# Autodesk Inventor assembly: DoubleCross_Rturn
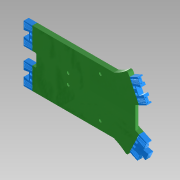
[picture p0: Inventor's stored thumbnail of the model, 180x180]
Saved by Autodesk Inventor 2021 (Build 250183000, 183)
## iProperties
Created: 2021-03-02
Part Number: DoubleCross_Rturn
Document SubType Name: Assembly
Designer: kumagai
Author: kumagai
## Documents named in this file (9)
- X:\Develop\CAD\PlaRails\DoubleCross\DoubleCross_SymWiden.iam
- X:\Develop\CAD\PlaRails\DoubleCross\DoubleCross\DoubleCross-ST_R.ipt
- Z:\Develop\CAD\PlaRails\DoubleCross.ipt
- X:\Develop\CAD\PlaRails\DoubleCross\DoubleCross\DoubleCross-ST_M.ipt
- X:\Develop\CAD\PlaRails\RailJointFemale.ipt
- X:\Develop\CAD\PlaRails\DoubleCross\DoubleCross\DoubleCross-SL_M.ipt
- X:\Develop\CAD\PlaRails\DoubleCross\DoubleCross.ipt
- X:\Develop\CAD\PlaRails\DoubleCross\DoubleCross\DoubleCross-SL_R.ipt
- X:\Develop\CAD\PlaRails\RailJointMale.ipt
## Components (8 placed, 6 different names)
1. Rail_LF — メイト:6, フラッシュ:12, フラッシュ:18
2. Rail_RF — メイト:5, フラッシュ:26, フラッシュ:15, フラッシュ:22, フラッシュ:23, フラッシュ:19
3. Rail_LB — フラッシュ:9, メイト:7, フラッシュ:11, フラッシュ:16, フラッシュ:20, フラッシュ:21
4. Rail_RB — フラッシュ:7, メイト:4, フラッシュ:14, フラッシュ:17, フラッシュ:24, フラッシュ:25
5. RailJointFemale:4 — メイト:5, フラッシュ:26, フラッシュ:19
6. RailJointMale:1 — フラッシュ:7, メイト:4, フラッシュ:14
7. RailJointFemale:1 — メイト:6, フラッシュ:12, フラッシュ:18
8. RailJointFemale:2 — フラッシュ:9, メイト:7, フラッシュ:11
## Relationships (21: Flush 17, Mate 4)
- フラッシュ:7 [Flush]: Rail_RB ↔ RailJointMale:1
- フラッシュ:9 [Flush]: Rail_LB ↔ RailJointFemale:2
- メイト:4 [Mate]: Rail_RB ↔ RailJointMale:1
- メイト:5 [Mate]: Rail_RF ↔ RailJointFemale:4
- メイト:6 [Mate]: Rail_LF ↔ RailJointFemale:1
- メイト:7 [Mate]: Rail_LB ↔ RailJointFemale:2
- フラッシュ:11 [Flush]: Rail_LB ↔ RailJointFemale:2
- フラッシュ:12 [Flush]: Rail_LF ↔ RailJointFemale:1
- フラッシュ:26 [Flush]: Rail_RF ↔ RailJointFemale:4
- フラッシュ:14 [Flush]: Rail_RB ↔ RailJointMale:1
- フラッシュ:15 [Flush]: Rail_RF
- フラッシュ:22 [Flush]: Rail_RF
- フラッシュ:23 [Flush]: Rail_RF
- フラッシュ:16 [Flush]: Rail_LB
- フラッシュ:17 [Flush]: Rail_RB
- フラッシュ:24 [Flush]: Rail_RB
- フラッシュ:25 [Flush]: Rail_RB
- フラッシュ:18 [Flush]: Rail_LF ↔ RailJointFemale:1
- フラッシュ:19 [Flush]: Rail_RF ↔ RailJointFemale:4
- フラッシュ:20 [Flush]: Rail_LB
- フラッシュ:21 [Flush]: Rail_LB
